# Autodesk Inventor assembly: Clamp with Piston Assembly
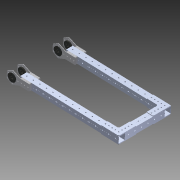
[picture p0: Inventor's stored thumbnail of the model, 180x180]
Saved by Autodesk Inventor 2014 (Build 180170000, 170)
## iProperties
Created: 2014-01-12
Part Number: Clamp with Piston Assembly
Document SubType Name: Assembly
Designer: Michael
Mass: 675.185 g
Surface Area: 3066.09 cm^2
Volume: 214.677 cm^3
Density: 3.14511 g/cm^3
Author: Michael
## Documents named in this file (7)
- C:\Users\Michael\Documents\GitHub\2014buildCAD\New Collector\Clamp with Piston Assembly.iam
- C:\Users\Michael\Documents\GitHub\2014buildCAD\New Collector\Vex Pro 1x1 rectangular tubing 14 in length.ipt
- C:\Users\Michael\Documents\GitHub\2014buildCAD\New Collector\Vex Pro 90 degree gusset.ipt
- C:\Users\Michael\Documents\GitHub\2014buildCAD\New Collector\Vex Pro End Bearing Mount.ipt
- C:\Users\Michael\Documents\GitHub\2014buildCAD\New Collector\Bearing Mount Spacer 1-8 in.ipt
- C:\Users\Michael\Documents\GitHub\2014buildCAD\New Collector\Vex Pro 1x1 rectangular tubing 6 in length.ipt
- C:\Users\Michael\Documents\GitHub\2014buildCAD\New Collector\Hex Bearing 3-8 in (FR6ZZL-hex (am-0692)).ipt
## Components (23 placed, 6 different names)
1. Vex Pro 1x1 rectangular tubing 14 in length:1 — Mate:23, Mate:26, Mate:40, Mate:41, Mate:42, Mate:43, Mate:128, Mate:129, Mate:130, Mate:131, Mate:132, Mate:133
2. Vex Pro 1x1 rectangular tubing 14 in length:2 — Mate:39, Mate:44, Mate:108, Mate:109, Mate:150, Mate:151, Mate:152, Mate:153, Mate:154, Mate:155, Mate:165
3. Vex Pro 90 degree gusset:1 — Mate:39, Mate:108, Mate:109, Mate:110, Mate:111, Mate:112
4. Vex Pro 90 degree gusset:2 — Mate:23, Mate:40, Mate:41, Mate:118
5. Vex Pro 90 degree gusset:3 — Mate:26, Mate:42, Mate:43, Mate:116, Mate:117
6. Vex Pro 90 degree gusset:4 — Mate:44, Mate:164, Mate:165
7. Vex Pro End Bearing Mount:3 — Mate:88, Mate:89, Mate:90, Mate:162, Mate:163
8. Vex Pro End Bearing Mount:4 — Mate:85, Mate:86, Mate:87, Mate:160, Mate:161
9. Bearing Mount Spacer 1-8 in:1 — Mate:85, Mate:86, Mate:87, Mate:125, Mate:126, Mate:127
10. Bearing Mount Spacer 1-8 in:2 — Mate:88, Mate:89, Mate:90, Mate:122, Mate:123, Mate:124
11. Vex Pro 1x1 rectangular tubing 6 in length:2 — Mate:110, Mate:111, Mate:112, Mate:116, Mate:117, Mate:118, Mate:164
12. Bearing Mount Spacer 1-8 in:5 — Mate:122, Mate:123, Mate:124, Mate:128, Mate:129, Mate:130
13. Bearing Mount Spacer 1-8 in:6 — Mate:125, Mate:126, Mate:127, Mate:131, Mate:132, Mate:133
14. Vex Pro End Bearing Mount:5 — Mate:158, Mate:159
15. Bearing Mount Spacer 1-8 in:7
16. Bearing Mount Spacer 1-8 in:8 — Mate:153, Mate:154, Mate:155
17. Vex Pro End Bearing Mount:6 — Mate:156, Mate:157
18. Bearing Mount Spacer 1-8 in:9
19. Bearing Mount Spacer 1-8 in:10 — Mate:150, Mate:151, Mate:152
20. Hex Bearing 3-8 in (FR6ZZL-hex (am-0692)):1 — Mate:160, Mate:161
21. Hex Bearing 3-8 in (FR6ZZL-hex (am-0692)):2 — Mate:162, Mate:163
22. Hex Bearing 3-8 in (FR6ZZL-hex (am-0692)):3 — Mate:156, Mate:157
23. Hex Bearing 3-8 in (FR6ZZL-hex (am-0692)):4 — Mate:158, Mate:159
## Relationships (62: Mate 62)
- Mate:23: Vex Pro 1x1 rectangular tubing 14 in length:1 ↔ Vex Pro 90 degree gusset:2
- Mate:26: Vex Pro 1x1 rectangular tubing 14 in length:1 ↔ Vex Pro 90 degree gusset:3
- Mate:39: Vex Pro 1x1 rectangular tubing 14 in length:2 ↔ Vex Pro 90 degree gusset:1
- Mate:40: Vex Pro 1x1 rectangular tubing 14 in length:1 ↔ Vex Pro 90 degree gusset:2
- Mate:41: Vex Pro 1x1 rectangular tubing 14 in length:1 ↔ Vex Pro 90 degree gusset:2
- Mate:42: Vex Pro 1x1 rectangular tubing 14 in length:1 ↔ Vex Pro 90 degree gusset:3
- Mate:43: Vex Pro 1x1 rectangular tubing 14 in length:1 ↔ Vex Pro 90 degree gusset:3
- Mate:44: Vex Pro 1x1 rectangular tubing 14 in length:2 ↔ Vex Pro 90 degree gusset:4
- Mate:85: Vex Pro End Bearing Mount:4 ↔ Bearing Mount Spacer 1-8 in:1
- Mate:86: Vex Pro End Bearing Mount:4 ↔ Bearing Mount Spacer 1-8 in:1
- Mate:87: Vex Pro End Bearing Mount:4 ↔ Bearing Mount Spacer 1-8 in:1
- Mate:88: Vex Pro End Bearing Mount:3 ↔ Bearing Mount Spacer 1-8 in:2
- Mate:89: Vex Pro End Bearing Mount:3 ↔ Bearing Mount Spacer 1-8 in:2
- Mate:90: Vex Pro End Bearing Mount:3 ↔ Bearing Mount Spacer 1-8 in:2
- Mate:108: Vex Pro 1x1 rectangular tubing 14 in length:2 ↔ Vex Pro 90 degree gusset:1
- Mate:109: Vex Pro 1x1 rectangular tubing 14 in length:2 ↔ Vex Pro 90 degree gusset:1
- Mate:110: Vex Pro 90 degree gusset:1 ↔ Vex Pro 1x1 rectangular tubing 6 in length:2
- Mate:111: Vex Pro 90 degree gusset:1 ↔ Vex Pro 1x1 rectangular tubing 6 in length:2
- Mate:112: Vex Pro 90 degree gusset:1 ↔ Vex Pro 1x1 rectangular tubing 6 in length:2
- Mate:116: Vex Pro 90 degree gusset:3 ↔ Vex Pro 1x1 rectangular tubing 6 in length:2
- Mate:117: Vex Pro 90 degree gusset:3 ↔ Vex Pro 1x1 rectangular tubing 6 in length:2
- Mate:118: Vex Pro 90 degree gusset:2 ↔ Vex Pro 1x1 rectangular tubing 6 in length:2
- Mate:122: Bearing Mount Spacer 1-8 in:2 ↔ Bearing Mount Spacer 1-8 in:5
- Mate:123: Bearing Mount Spacer 1-8 in:2 ↔ Bearing Mount Spacer 1-8 in:5
- Mate:124: Bearing Mount Spacer 1-8 in:2 ↔ Bearing Mount Spacer 1-8 in:5
- Mate:125: Bearing Mount Spacer 1-8 in:1 ↔ Bearing Mount Spacer 1-8 in:6
- Mate:126: Bearing Mount Spacer 1-8 in:1 ↔ Bearing Mount Spacer 1-8 in:6
- Mate:127: Bearing Mount Spacer 1-8 in:1 ↔ Bearing Mount Spacer 1-8 in:6
- Mate:128: Vex Pro 1x1 rectangular tubing 14 in length:1 ↔ Bearing Mount Spacer 1-8 in:5
- Mate:129: Vex Pro 1x1 rectangular tubing 14 in length:1 ↔ Bearing Mount Spacer 1-8 in:5
- Mate:130: Vex Pro 1x1 rectangular tubing 14 in length:1 ↔ Bearing Mount Spacer 1-8 in:5
- Mate:131: Vex Pro 1x1 rectangular tubing 14 in length:1 ↔ Bearing Mount Spacer 1-8 in:6
- Mate:132: Vex Pro 1x1 rectangular tubing 14 in length:1 ↔ Bearing Mount Spacer 1-8 in:6
- Mate:133: Vex Pro 1x1 rectangular tubing 14 in length:1 ↔ Bearing Mount Spacer 1-8 in:6
- [Mate]: Vex Pro End Bearing Mount:5 ↔ Bearing Mount Spacer 1-8 in:7
- [Mate]: Vex Pro End Bearing Mount:5 ↔ Bearing Mount Spacer 1-8 in:7
- [Mate]: Vex Pro End Bearing Mount:5 ↔ Bearing Mount Spacer 1-8 in:7
- [Mate]: Bearing Mount Spacer 1-8 in:7 ↔ Bearing Mount Spacer 1-8 in:8
- [Mate]: Bearing Mount Spacer 1-8 in:7 ↔ Bearing Mount Spacer 1-8 in:8
- [Mate]: Bearing Mount Spacer 1-8 in:7 ↔ Bearing Mount Spacer 1-8 in:8
- [Mate]: Vex Pro End Bearing Mount:6 ↔ Bearing Mount Spacer 1-8 in:9
- [Mate]: Vex Pro End Bearing Mount:6 ↔ Bearing Mount Spacer 1-8 in:9
- [Mate]: Vex Pro End Bearing Mount:6 ↔ Bearing Mount Spacer 1-8 in:9
- [Mate]: Bearing Mount Spacer 1-8 in:9 ↔ Bearing Mount Spacer 1-8 in:10
- [Mate]: Bearing Mount Spacer 1-8 in:9 ↔ Bearing Mount Spacer 1-8 in:10
- [Mate]: Bearing Mount Spacer 1-8 in:9 ↔ Bearing Mount Spacer 1-8 in:10
- Mate:150: Vex Pro 1x1 rectangular tubing 14 in length:2 ↔ Bearing Mount Spacer 1-8 in:10
- Mate:151: Vex Pro 1x1 rectangular tubing 14 in length:2 ↔ Bearing Mount Spacer 1-8 in:10
- Mate:152: Vex Pro 1x1 rectangular tubing 14 in length:2 ↔ Bearing Mount Spacer 1-8 in:10
- Mate:153: Vex Pro 1x1 rectangular tubing 14 in length:2 ↔ Bearing Mount Spacer 1-8 in:8
- Mate:154: Vex Pro 1x1 rectangular tubing 14 in length:2 ↔ Bearing Mount Spacer 1-8 in:8
- Mate:155: Vex Pro 1x1 rectangular tubing 14 in length:2 ↔ Bearing Mount Spacer 1-8 in:8
- Mate:156: Vex Pro End Bearing Mount:6 ↔ Hex Bearing 3-8 in (FR6ZZL-hex (am-0692)):3
- Mate:157: Vex Pro End Bearing Mount:6 ↔ Hex Bearing 3-8 in (FR6ZZL-hex (am-0692)):3
- Mate:158: Vex Pro End Bearing Mount:5 ↔ Hex Bearing 3-8 in (FR6ZZL-hex (am-0692)):4
- Mate:159: Vex Pro End Bearing Mount:5 ↔ Hex Bearing 3-8 in (FR6ZZL-hex (am-0692)):4
- Mate:160: Vex Pro End Bearing Mount:4 ↔ Hex Bearing 3-8 in (FR6ZZL-hex (am-0692)):1
- Mate:161: Vex Pro End Bearing Mount:4 ↔ Hex Bearing 3-8 in (FR6ZZL-hex (am-0692)):1
- Mate:162: Vex Pro End Bearing Mount:3 ↔ Hex Bearing 3-8 in (FR6ZZL-hex (am-0692)):2
- Mate:163: Vex Pro End Bearing Mount:3 ↔ Hex Bearing 3-8 in (FR6ZZL-hex (am-0692)):2
- Mate:164: Vex Pro 90 degree gusset:4 ↔ Vex Pro 1x1 rectangular tubing 6 in length:2
- Mate:165: Vex Pro 1x1 rectangular tubing 14 in length:2 ↔ Vex Pro 90 degree gusset:4
## Named parameters: d167_d158 = 0 mm, d168_d159 = 0 mm, d169_d160 = 0 mm, d172_d118 = 0 mm, d173_d119 = 0 mm, d174_d120 = 0 mm, d175_d158 = 0 mm, d176_d159 = 0 mm, d177_d160 = 0 mm, d180_d118 = 0 mm, d181_d119 = 0 mm, d182_d120 = 0 mm
